# Autodesk Inventor assembly: assembly
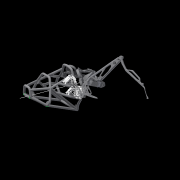
[picture p0: Inventor's stored thumbnail of the model, 180x180]
Saved by Autodesk Inventor 2020 (Build 240168000, 168)
## iProperties
Created: 2020-03-24
Part Number: assembly
Document SubType Name: Assembly
Designer: valer
Author: valer
## Documents named in this file (13)
- C:\Users\valer\Desktop\drummingrobot\src\Robot.iam
- C:\Users\valer\Desktop\drummingrobot\src\Chest.ipt
- C:\Users\valer\Desktop\drummingrobot\src\HeadScaled.ipt
- C:\Users\valer\Desktop\drummingrobot\src\UpperArmServoDynamixelXM430-W350-T.ipt
- C:\Users\valer\Desktop\drummingrobot\src\Forearm.ipt
- C:\Users\valer\Desktop\drummingrobot\src\UpperArm.ipt
- C:\Users\valer\Desktop\drummingrobot\src\UpperArmBracket.ipt
- C:\Users\valer\Desktop\drummingrobot\src\UpperArmMount.ipt
- C:\Users\valer\Desktop\drummingrobot\src\ShoulderBracket.ipt
- C:\Users\valer\Desktop\drummingrobot\src\ShoulderChestBracket.ipt
- C:\Users\valer\Desktop\drummingrobot\src\external\ShoulderConnectingRod.ipt
- C:\Users\valer\Desktop\drummingrobot\src\external\RodEnd.ipt
- C:\Users\valer\Desktop\drummingrobot\src\external\RodEndBall.ipt
## Components (32 placed, 12 different names)
1. Chest:1 — Angle:1, Angle:4, Flush:2, Mate:54, Mate:55, Angle:6, Mate:57, Mate:58
2. HeadScaled:1 — Angle:6
3. UpperArmServoDynamixelXM430-W350-T:1 — Angle:1, Mate:10, Mate:11, Mate:12, Mate:13, Mate:14, Angle:2, Mate:15
4. Forearm:1 — Mate:1, Flush:1
5. UpperArm:1 — Mate:1, Flush:1, Mate:2, Mate:3, Mate:4, Mate:5
6. UpperArmBracket:1 — Mate:2, Mate:3, Mate:6, Mate:8, Mate:25
7. UpperArmMount:1 — Mate:6, Mate:7, Mate:8, Mate:10, Mate:11, Angle:3, Angle:5, Mate:25
8. UpperArmBracket:2 — Mate:4, Mate:5, Mate:7
9. ShoulderBracket:1 — Mate:12, Mate:14, Angle:2, Mate:46, Mate:47
10. ShoulderBracket:2 — Mate:13, Mate:15, Angle:3, Mate:52, Mate:53
11. ShoulderChestBracket:1 — Angle:4, Angle:5, Mate:48, Mate:49, Mate:50, Mate:51, Flush:2, Mate:54, Mate:55
12. ChestConnectingRod:1 — Mate:17, Mate:19, Mate:20
13. ChestConnectingRod:2 — Mate:26, Mate:27, Mate:28, Mate:56
14. ChestConnectingRod:3 — Mate:40, Mate:42, Mate:43
15. ChestConnectingRod:4 — Mate:34, Mate:35, Mate:36
16. RodEnd:1 — Mate:19, Mate:20, Mate:32
17. RodEnd:2 — Mate:17, Mate:30, Mate:46
18. RodEnd:3 — Mate:26, Mate:27, Mate:31, Mate:47
19. RodEnd:4 — Mate:28, Mate:33, Mate:56
20. RodEndBall:5 — Mate:30
21. RodEndBall:6 — Mate:33, Mate:49
22. RodEndBall:7 — Mate:31
23. RodEndBall:8 — Mate:32, Mate:48
24. RodEnd:5 — Mate:35, Mate:36, Mate:39
25. RodEnd:6 — Mate:42, Mate:43, Mate:45
26. RodEnd:7 — Mate:34, Mate:38
27. RodEnd:8 — Mate:40, Mate:44, Mate:53
28. RodEndBall:9 — Mate:39, Mate:50
29. RodEndBall:10 — Mate:45, Mate:51
30. RodEndBall:11 — Mate:38, Mate:52
31. RodEndBall:12 — Mate:44
32. ShoulderChestBracket:2 — Mate:57, Mate:58
## Relationships (56: Mate 48, Angle 6, Flush 2)
- Angle:1 (0 deg): Chest:1 ↔ UpperArmServoDynamixelXM430-W350-T:1
- Mate:1: Forearm:1 ↔ UpperArm:1
- Flush:1 (12.7 mm): Forearm:1 ↔ UpperArm:1
- Mate:2: UpperArm:1 ↔ UpperArmBracket:1
- Mate:3: UpperArm:1 ↔ UpperArmBracket:1
- Mate:4: UpperArm:1 ↔ UpperArmBracket:2
- Mate:5: UpperArm:1 ↔ UpperArmBracket:2
- Mate:6: UpperArmBracket:1 ↔ UpperArmMount:1
- Mate:7: UpperArmMount:1 ↔ UpperArmBracket:2
- Mate:8: UpperArmBracket:1 ↔ UpperArmMount:1
- Mate:10: UpperArmServoDynamixelXM430-W350-T:1 ↔ UpperArmMount:1
- Mate:11: UpperArmServoDynamixelXM430-W350-T:1 ↔ UpperArmMount:1
- Mate:12: UpperArmServoDynamixelXM430-W350-T:1 ↔ ShoulderBracket:1
- Mate:13: UpperArmServoDynamixelXM430-W350-T:1 ↔ ShoulderBracket:2
- Mate:14: UpperArmServoDynamixelXM430-W350-T:1 ↔ ShoulderBracket:1
- Angle:2 (0 deg): UpperArmServoDynamixelXM430-W350-T:1 ↔ ShoulderBracket:1
- Mate:15: UpperArmServoDynamixelXM430-W350-T:1 ↔ ShoulderBracket:2
- Angle:3 (0 deg): UpperArmMount:1 ↔ ShoulderBracket:2
- Angle:4 (0 deg): Chest:1 ↔ ShoulderChestBracket:1
- Mate:17: ChestConnectingRod:1 ↔ RodEnd:2
- Mate:19: ChestConnectingRod:1 ↔ RodEnd:1
- Mate:20 (-25.4 mm): ChestConnectingRod:1 ↔ RodEnd:1
- Angle:5 (0 deg): UpperArmMount:1 ↔ ShoulderChestBracket:1
- Mate:25 (12.7 mm): UpperArmBracket:1 ↔ UpperArmMount:1
- Mate:26: ChestConnectingRod:2 ↔ RodEnd:3
- Mate:27 (-25.4 mm): ChestConnectingRod:2 ↔ RodEnd:3
- Mate:28: ChestConnectingRod:2 ↔ RodEnd:4
- Mate:30: RodEnd:2 ↔ RodEndBall:5
- Mate:31: RodEnd:3 ↔ RodEndBall:7
- Mate:32: RodEnd:1 ↔ RodEndBall:8
- Mate:33: RodEnd:4 ↔ RodEndBall:6
- Mate:34: ChestConnectingRod:4 ↔ RodEnd:7
- Mate:35: ChestConnectingRod:4 ↔ RodEnd:5
- Mate:36 (-25.4 mm): ChestConnectingRod:4 ↔ RodEnd:5
- Mate:38: RodEnd:7 ↔ RodEndBall:11
- Mate:39: RodEnd:5 ↔ RodEndBall:9
- Mate:40: ChestConnectingRod:3 ↔ RodEnd:8
- Mate:42: ChestConnectingRod:3 ↔ RodEnd:6
- Mate:43 (-25.4 mm): ChestConnectingRod:3 ↔ RodEnd:6
- Mate:44: RodEnd:8 ↔ RodEndBall:12
- Mate:45: RodEnd:6 ↔ RodEndBall:10
- Mate:46: ShoulderBracket:1 ↔ RodEnd:2
- Mate:47: ShoulderBracket:1 ↔ RodEnd:3
- Mate:48: ShoulderChestBracket:1 ↔ RodEndBall:8
- Mate:49: ShoulderChestBracket:1 ↔ RodEndBall:6
- Mate:50: ShoulderChestBracket:1 ↔ RodEndBall:9
- Mate:51: ShoulderChestBracket:1 ↔ RodEndBall:10
- Mate:52: ShoulderBracket:2 ↔ RodEndBall:11
- Mate:53: ShoulderBracket:2 ↔ RodEnd:8
- Flush:2: Chest:1 ↔ ShoulderChestBracket:1
- Mate:54 (10.16 mm): Chest:1 ↔ ShoulderChestBracket:1
- Mate:55: Chest:1 ↔ ShoulderChestBracket:1
- Mate:56 (-25.4 mm): ChestConnectingRod:2 ↔ RodEnd:4
- Angle:6 (0 deg): Chest:1 ↔ HeadScaled:1
- Mate:57 (10.16 mm): Chest:1 ↔ ShoulderChestBracket:2
- Mate:58: Chest:1 ↔ ShoulderChestBracket:2
